# Autodesk Inventor assembly: grabber claw
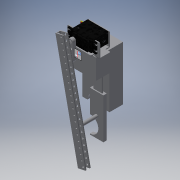
[picture p0: Inventor's stored thumbnail of the model, 180x180]
Saved by Autodesk Inventor 2019 (Build 230136000, 136)
## iProperties
Created: 2020-10-24
Part Number: grabber claw
Document SubType Name: Assembly
Designer: User
Author: User
## Documents named in this file (8)
- C:\Robotics\CAD\2020-21-CAD\grabber\grabber claw.iam
- C:\Robotics\CAD\2020-21-CAD\custom parts\graber base.ipt
- C:\Robotics\CAD\2020-21-CAD\custom parts\hook.ipt
- C:\Robotics\CAD\COTSParts\Tetrix\Tetrix bracket - single servo.ipt
- C:\Robotics\CAD\COTSParts\Tetrix\Tetrix 180 Servo.ipt
- C:\Robotics\CAD\COTSParts\Actobotics\585 parts\585396MiniChannel8in.ipt
- 585396MiniChannel8in.ipt
- C:\Robotics\CAD\COTSParts\Actobotics\525 parts\525116.ipt
## Components (6 placed, 6 different names)
1. graber base:1 — Mate:1, Flush:1, Mate:5, Flush:3, Flush:4
2. hook:1 — Mate:1, Flush:1, Mate:12
3. Tetrix bracket - single servo:1 — Mate:3, Mate:4, Flush:2, Mate:5, Flush:3, Flush:4
4. Tetrix 180 Servo:1 — Mate:3, Mate:4, Flush:2, Mate:6, Mate:7
5. 585396MiniChannel8in:1 — Mate:8, Mate:11, Mate:12
6. 525116:1 — Mate:6, Mate:7, Mate:8, Mate:11
## Relationships (13: Mate 9, Flush 4)
- Mate:1: graber base:1 ↔ hook:1
- Flush:1 (-25.4 mm): graber base:1 ↔ hook:1
- Mate:3: Tetrix bracket - single servo:1 ↔ Tetrix 180 Servo:1
- Mate:4 (5.08 mm): Tetrix bracket - single servo:1 ↔ Tetrix 180 Servo:1
- Flush:2 (3.81 mm): Tetrix bracket - single servo:1 ↔ Tetrix 180 Servo:1
- Mate:5: graber base:1 ↔ Tetrix bracket - single servo:1
- Flush:3: graber base:1 ↔ Tetrix bracket - single servo:1
- Flush:4 (-6.35 mm): graber base:1 ↔ Tetrix bracket - single servo:1
- Mate:6: Tetrix 180 Servo:1 ↔ 525116:1
- Mate:7: Tetrix 180 Servo:1 ↔ 525116:1
- Mate:8: 585396MiniChannel8in:1 ↔ 525116:1
- Mate:11: 585396MiniChannel8in:1 ↔ 525116:1
- Mate:12: hook:1 ↔ 585396MiniChannel8in:1
